# Autodesk Inventor assembly: Assembly1
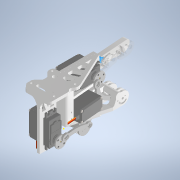
[picture p0: Inventor's stored thumbnail of the model, 180x180]
Saved by Autodesk Inventor 2020.3 (Build 243373000, 373)
## iProperties
Created: 2021-04-08
Part Number: Assembly1
Document SubType Name: Assembly
Designer: sanyi
Author: sanyi
## Documents named in this file (19)
- E:\Dokumentumok\Simonyi\INDACT\Robotarm - kézfej fileok\Assembly1.iam
- E:\Dokumentumok\Simonyi\INDACT\Robotarm - kézfej fileok\kéz12.0\Solid1_1_v2.ipt
- E:\Dokumentumok\Simonyi\INDACT\Robotarm - kézfej fileok\kéz12.0\Solid3_1v2.ipt
- E:\Dokumentumok\Simonyi\INDACT\Robotarm - kézfej fileok\kéz12.0\Solid1.ipt
- E:\Dokumentumok\Simonyi\INDACT\Robotarm - kézfej fileok\kéz12.0\Solid1_MIR1.ipt
- E:\Dokumentumok\Simonyi\INDACT\Robotarm - kézfej fileok\kéz12.0\Solid2.ipt
- E:\Dokumentumok\Simonyi\INDACT\Robotarm - kézfej fileok\kéz12.0\Solid2_MIR2.ipt
- E:\Dokumentumok\Simonyi\INDACT\Robotarm - kézfej fileok\kéz12.0\Solid3.ipt
- E:\Dokumentumok\Simonyi\INDACT\Robotarm - kézfej fileok\kéz12.0\Solid3_MIR2.ipt
- E:\Dokumentumok\Simonyi\INDACT\Robotarm - kézfej fileok\kéz12.0\Solid5.ipt
- E:\Dokumentumok\Simonyi\INDACT\Robotarm - kézfej fileok\kéz12.0\Solid6.ipt
- E:\Dokumentumok\Simonyi\INDACT\Robotarm - kézfej fileok\kéz12.0\Solid1_11.ipt
- E:\Dokumentumok\Simonyi\INDACT\Robotarm - kézfej fileok\kéz12.0\Solid2_1.ipt
- E:\Dokumentumok\Simonyi\INDACT\Robotarm - kézfej fileok\kéz12.0\Part2.ipt
- E:\Dokumentumok\Simonyi\INDACT\Robotarm - kézfej fileok\kéz12.0\Part3.ipt
- E:\Dokumentumok\Simonyi\INDACT\Robotarm - kézfej fileok\kéz12.0\Part6.ipt
- E:\Dokumentumok\Simonyi\INDACT\Robotarm - kézfej fileok\kéz12.0\tower-pro-mg-995-analog-servo-1.snapshot.18\TOWER PRO MG-995, ANALOG SERVO.iam
- E:\Dokumentumok\Simonyi\INDACT\Robotarm - kézfej fileok\kéz12.0\motortarcsa.ipt
- E:\Dokumentumok\Simonyi\INDACT\Robotarm - kézfej fileok\kéz12.0\Solid13_mother_m2_5.ipt
## Components (25 placed, 18 different names)
1. Solid1_1_v2:1 — Insert:1, Insert:2, Flush:1, Insert:49, Insert:64, Insert:65, Insert:66, Insert:85, Insert:87, Insert:88, Insert:89, Insert:90, Insert:91
2. Solid3_1v2:1 — Insert:1, Insert:2
3. Solid1:4 — Insert:91, Insert:92
4. Solid1_MIR1:4 — Insert:85, Insert:86, Insert:96
5. Solid5:4 — Insert:49, Insert:94
6. Solid6:4 — Insert:95
7. Solid1_11:1 — Insert:66, Insert:67, Insert:72, Insert:73, Mate:12
8. Solid2_1:1 — Insert:64, Insert:65, Insert:67, Insert:68, Insert:69, Insert:70, Insert:71, Mate:13
9. Part2:1 — Insert:86
10. Part3:1 — Insert:78
11. Part6:1 — Insert:80
12. TOWER PRO MG-995, ANALOG SERVO:1 [sub-assembly] — Insert:68, Insert:69, Insert:74
13. TOWER PRO MG-995, ANALOG SERVO:2 [sub-assembly] — Insert:70, Insert:71, Insert:76
14. TOWER PRO MG-995, ANALOG SERVO:3 [sub-assembly] — Insert:72, Insert:73, Insert:75
15. motortarcsa:1 — Insert:74, Insert:80
16. motortarcsa:2 — Insert:75
17. motortarcsa:3 — Insert:76, Insert:78
18. Solid13_mother_m2_5:1 — Insert:87
19. Solid13_mother_m2_5:2 — Insert:88
20. Solid13_mother_m2_5:3 — Insert:89
21. Solid13_mother_m2_5:4 — Insert:90
22. Solid2:1 — Insert:92, Insert:93, Insert:94, Angle:11
23. Solid2_MIR2:1 — Insert:96, Angle:11, Insert:97
24. Solid3:1 — Insert:93, Insert:95, Angle:12
25. Solid3_MIR2:1 — Insert:97, Angle:12
## Relationships (39: Insert 32, Mate 3, Angle 3, Flush 1)
- Insert:1: Solid1_1_v2:1 ↔ Solid3_1v2:1
- Insert:2: Solid1_1_v2:1 ↔ Solid3_1v2:1
- Flush:1: Solid1_1_v2:1
- [Mate]: Solid1:4 ↔ Solid1_MIR1:4
- [Angle] (0 deg): Solid1:4 ↔ Solid1_MIR1:4
- [Insert] (0.5 mm): Solid1:4 ↔ Solid6:4
- Insert:49 (0.5 mm): Solid1_1_v2:1 ↔ Solid5:4
- Insert:64: Solid1_1_v2:1 ↔ Solid2_1:1
- Insert:65: Solid1_1_v2:1 ↔ Solid2_1:1
- Insert:66: Solid1_1_v2:1 ↔ Solid1_11:1
- Insert:67: Solid1_11:1 ↔ Solid2_1:1
- Insert:68: Solid2_1:1 ↔ TOWER PRO MG-995, ANALOG SERVO:1
- Insert:69: Solid2_1:1 ↔ TOWER PRO MG-995, ANALOG SERVO:1
- Insert:70: Solid2_1:1 ↔ TOWER PRO MG-995, ANALOG SERVO:2
- Insert:71: Solid2_1:1 ↔ TOWER PRO MG-995, ANALOG SERVO:2
- Insert:72: Solid1_11:1 ↔ TOWER PRO MG-995, ANALOG SERVO:3
- Insert:73: Solid1_11:1 ↔ TOWER PRO MG-995, ANALOG SERVO:3
- Insert:74: TOWER PRO MG-995, ANALOG SERVO:1 ↔ motortarcsa:1
- Insert:75: TOWER PRO MG-995, ANALOG SERVO:3 ↔ motortarcsa:2
- Insert:76: TOWER PRO MG-995, ANALOG SERVO:2 ↔ motortarcsa:3
- Insert:78 (0.2 mm): Part3:1 ↔ motortarcsa:3
- Insert:80 (0.2 mm): Part6:1 ↔ motortarcsa:1
- Insert:85 (0.2 mm): Solid1_1_v2:1 ↔ Solid1_MIR1:4
- Insert:86 (1.876 mm): Solid1_MIR1:4 ↔ Part2:1
- Insert:87: Solid1_1_v2:1 ↔ Solid13_mother_m2_5:1
- Insert:88: Solid1_1_v2:1 ↔ Solid13_mother_m2_5:2
- Insert:89: Solid1_1_v2:1 ↔ Solid13_mother_m2_5:3
- Insert:90: Solid1_1_v2:1 ↔ Solid13_mother_m2_5:4
- Insert:91 (0.2 mm): Solid1_1_v2:1 ↔ Solid1:4
- Insert:92 (0.2 mm): Solid1:4 ↔ Solid2:1
- Insert:93 (0.2 mm): Solid2:1 ↔ Solid3:1
- Insert:94 (3.5 mm): Solid5:4 ↔ Solid2:1
- Insert:95 (3.5 mm): Solid6:4 ↔ Solid3:1
- Insert:96 (0.2 mm): Solid1_MIR1:4 ↔ Solid2_MIR2:1
- Angle:11 (0 deg): Solid2:1 ↔ Solid2_MIR2:1
- Insert:97 (0.2 mm): Solid2_MIR2:1 ↔ Solid3_MIR2:1
- Angle:12 (0 deg): Solid3:1 ↔ Solid3_MIR2:1
- Mate:12: Solid1_11:1
- Mate:13: Solid2_1:1
## Named parameters: d75_d24 = 0.5 mm, d81_d50 = 0 mm, d84_d53 = 0 deg
